# Autodesk Inventor assembly: body_top_v1
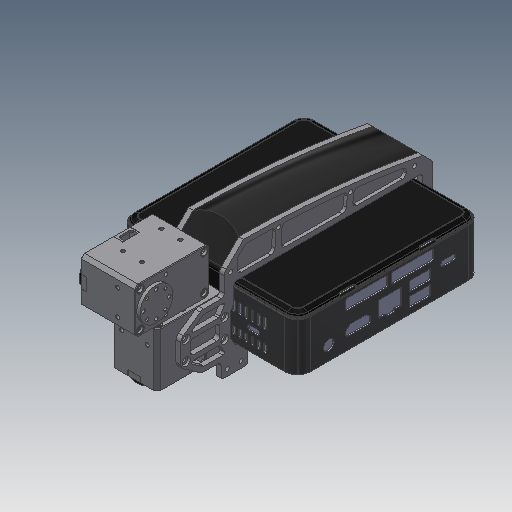
[picture p0: Inventor's stored thumbnail of the model, 512x512]
Saved by Autodesk Inventor 2019.4 (Build 234330000, 330)
## iProperties
Created: 2018-08-31
Part Number: body_top_v1
Material: 一般
Document SubType Name: Assembly
Designer: student
Author: student
## Documents named in this file (7)
- C:\Workspace\Yunit8-HaptHexa\Hardware\Inventor\Computer\_Computer.iam
- C:\Workspace\Yunit8-HaptHexa\Hardware\Inventor\X430\XL-430.iam
- C:\Workspace\Yunit8-HaptHexa\Hardware\Inventor\Computer\NUC7i5-7BNK-CHASSIS.ipt
- C:\Workspace\Yunit8-HaptHexa\Hardware\Inventor\Computer\VerticalFrame.ipt
- C:\Workspace\Yunit8-HaptHexa\Hardware\Inventor\Computer\VerticalFrame_mir.ipt
- C:\Workspace\Yunit8-HaptHexa\Hardware\Inventor\Computer\Handler.ipt
- C:\Workspace\Yunit8-HaptHexa\Hardware\Inventor\Computer\NUC_tab.ipt
## Components (7 placed, 6 different names)
1. NUC7i5-7BNK-CHASSIS:1 — メイト:38, メイト:44, フラッシュ:9, メイト:45, フラッシュ:12
2. XL-430:1 [sub-assembly] — フラッシュ:6, メイト:41
3. XL-430:2 [sub-assembly] — メイト:38, メイト:40, メイト:41, メイト:43, メイト:46
4. VerticalFrame:1 — フラッシュ:7, フラッシュ:8, メイト:43
5. VerticalFrame_mir:1 — メイト:47, フラッシュ:10
6. Handler:1 — フラッシュ:11
7. NUC_tab:1 — フラッシュ:12
## Relationships (15: Mate 8, Flush 7)
- メイト:38 [Mate]: NUC7i5-7BNK-CHASSIS:1 ↔ XL-430:2
- メイト:40 [Mate]: XL-430:2
- フラッシュ:6 [Flush]: XL-430:1
- メイト:41 [Mate] (3 mm): XL-430:1 ↔ XL-430:2
- フラッシュ:7 [Flush]: VerticalFrame:1
- フラッシュ:8 [Flush]: VerticalFrame:1
- メイト:43 [Mate]: XL-430:2 ↔ VerticalFrame:1
- メイト:44 [Mate]: NUC7i5-7BNK-CHASSIS:1
- フラッシュ:9 [Flush]: NUC7i5-7BNK-CHASSIS:1
- メイト:45 [Mate]: NUC7i5-7BNK-CHASSIS:1
- メイト:46 [Mate] (-5 mm): XL-430:2
- メイト:47 [Mate]: VerticalFrame_mir:1
- フラッシュ:10 [Flush]: VerticalFrame_mir:1
- フラッシュ:11 [Flush]: Handler:1
- フラッシュ:12 [Flush]: NUC7i5-7BNK-CHASSIS:1 ↔ NUC_tab:1
